# Autodesk Inventor assembly: Assembly
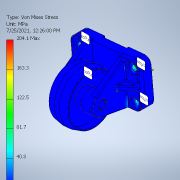
[picture p0: Inventor's stored thumbnail of the model, 180x180]
Saved by Autodesk Inventor 2020 (Build 240168000, 168)
## iProperties
Created: 2021-06-13
Part Number: Assembly
Document SubType Name: Assembly
Designer: joelm
Mass: 3411.09 g
Surface Area: 1161.28 cm^2
Volume: 474.513 cm^3
Density: 7.18861 g/cm^3
Author: joelm
## Documents named in this file (12)
- D:\Carreer 4.1\Manufacturing Tech\CasterWheel\Assembly.iam
- D:\Carreer 4.1\Manufacturing Tech\CasterWheel\axle.ipt
- D:\Carreer 4.1\Manufacturing Tech\CasterWheel\axleSupport.ipt
- D:\Carreer 4.1\Manufacturing Tech\CasterWheel\topPlate.ipt
- D:\Carreer 4.1\Manufacturing Tech\CasterWheel\wheel.ipt
- D:\Carreer 4.1\Manufacturing Tech\CasterWheel\axleSupport2\axleSupportMirror.ipt
- D:\Carreer 4.1\Manufacturing Tech\CasterWheel\Assembly\AIP\FEA\doecl87j4.fins
- D:\Carreer 4.1\Manufacturing Tech\CasterWheel\Assembly\AIP\FEA\doecl87k0.fsat
- D:\Carreer 4.1\Manufacturing Tech\CasterWheel\Assembly\AIP\FEA\doecl87k0.ftes
- D:\Carreer 4.1\Manufacturing Tech\CasterWheel\Assembly\AIP\FEA\doecl87k0.fwiz
- D:\Carreer 4.1\Manufacturing Tech\CasterWheel\Assembly\AIP\FEA\doecl885c.fmsh
- D:\Carreer 4.1\Manufacturing Tech\CasterWheel\Assembly\AIP\FEA\doecl8868.fres
## Components (5 placed, 5 different names)
1. axle:1 — Mate:1, Mate:2, Flush:1
2. axleSupport:1 — Mate:2, Flush:1, Mate:4, Mate:6, Mate:7, Flush:2
3. topPlate:1 — Mate:6, Mate:7, Flush:2, Mate:8, Mate:9
4. wheel:1 — Mate:1, Mate:4, Mate:10
5. axleSupportMirror:1 — Mate:8, Mate:9, Mate:10
## Relationships (10: Mate 8, Flush 2)
- Mate:1: axle:1 ↔ wheel:1
- Mate:2: axle:1 ↔ axleSupport:1
- Flush:1 (-2 mm): axle:1 ↔ axleSupport:1
- Mate:4: axleSupport:1 ↔ wheel:1
- Mate:6: axleSupport:1 ↔ topPlate:1
- Mate:7: axleSupport:1 ↔ topPlate:1
- Flush:2: axleSupport:1 ↔ topPlate:1
- Mate:8: topPlate:1 ↔ axleSupportMirror:1
- Mate:9: topPlate:1 ↔ axleSupportMirror:1
- Mate:10: wheel:1 ↔ axleSupportMirror:1
## Named parameters: sa_0 = 981, sa_1 = 1e+07
note: some values were not read from the file. Shown as the stored number, unit unknown: "sa_0", "sa_1".
